# Autodesk Inventor assembly: 高速轴
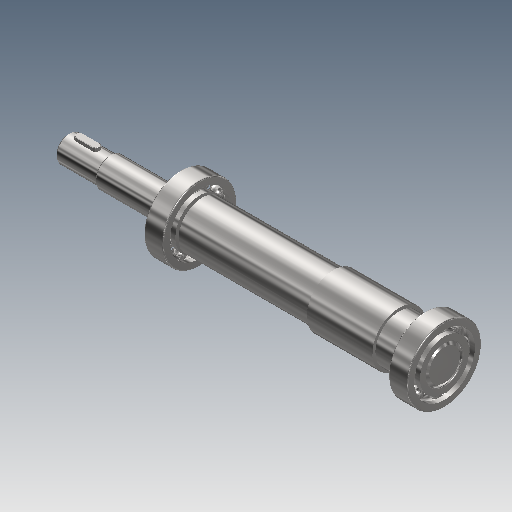
[picture p0: Inventor's stored thumbnail of the model, 512x512]
Saved by Autodesk Inventor 2025 (Build 290162000, 162)
## iProperties
Created: 2025-03-05
Part Number: 高速轴
Document SubType Name: Assembly
Designer: liukan
Author: liukan
## Documents named in this file (6)
- D:\2025春夏那些过往\2025春夏课程文件\机械设计课程设计（甲）\Inventor files\高速轴.iam
- D:\2025春夏那些过往\2025春夏课程文件\机械设计课程设计（甲）\Inventor files\轴1.ipt
- D:\2025春夏那些过往\2025春夏课程文件\机械设计课程设计（甲）\Inventor files\高速轴\设计加速器\轴承1.iam
- D:\2025春夏那些过往\2025春夏课程文件\机械设计课程设计（甲）\Inventor files\高速轴\设计加速器\轴承2.iam
- D:\2025春夏那些过往\2025春夏课程文件\机械设计课程设计（甲）\Inventor files\高速轴\设计加速器\键联接1.iam
- D:\2025春夏那些过往\2025春夏课程文件\机械设计课程设计（甲）\Inventor files\高速轴\设计加速器\键联接2.iam
## Components (5 placed, 3 different names)
1. 轴:1 — 配合:1, 表面齐平:1, 配合:2, 配合:3, 表面齐平:2, 角度:1, 配合:4
2. 轴承:1 [sub-assembly] — 配合:1, 表面齐平:1
3. 轴承:2 [sub-assembly] — 配合:2, 配合:3
4. 键联接:1 [sub-assembly]
5. 键联接:2 [sub-assembly] — 表面齐平:2, 角度:1, 配合:4
## Relationships (7: Mate 4, Flush 2, Angle 1)
- 配合:1 [Mate]: 轴:1 ↔ 轴承:1
- 表面齐平:1 [Flush]: 轴:1 ↔ 轴承:1
- 配合:2 [Mate]: 轴:1 ↔ 轴承:2
- 配合:3 [Mate]: 轴:1 ↔ 轴承:2
- 表面齐平:2 [Flush] (7 mm): 轴:1 ↔ 键联接:2
- 角度:1 [Angle] (0 deg): 轴:1 ↔ 键联接:2
- 配合:4 [Mate]: 轴:1 ↔ 键联接:2
